# Autodesk Inventor assembly: Second Technological Stage Table Top Assembly
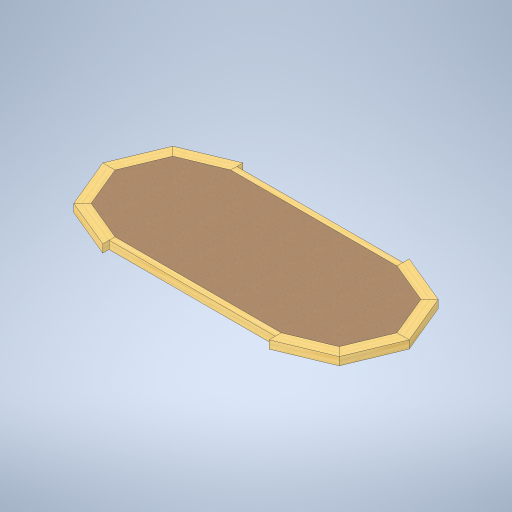
[picture p0: Inventor's stored thumbnail of the model, 512x512]
Saved by Autodesk Inventor 2024 (Build 280153000, 153)
## iProperties
Created: 2020-04-16
Part Number: Second Technological Stage Table Top Assembly
Document SubType Name: Assembly
Designer: SauliusD
Author: SauliusD
## Documents named in this file (4)
- C:\W4INV 2024 Design\PROJECTS\Samples\Composite Material Table\2 Technological Stage Table\Second Technological Stage Table Top Assembly.iam
- C:\W4INV 2024 Design\PROJECTS\Samples\Composite Material Table\2 Technological Stage Table\Round Frame.ipt
- C:\W4INV 2024 Design\PROJECTS\Samples\Composite Material Table\2 Technological Stage Table\Side Insert.ipt
- C:\W4INV 2024 Design\PROJECTS\Samples\Composite Material Table\1 Technolgical stage\First Technolgical stage Table Top Glued Assembly.ipt
## Components (11 placed, 3 different names)
1. Round Frame:1 — Mate:1, Mate:2
2. Side Insert:1
3. First Technolgical stage Table Top Glued Assembly:1 — Flush:1, Flush:2, Flush:3
4. Side Insert:2
5. Round Frame:2
6. Round Frame:3
7. Round Frame:4
8. Round Frame:5 — Mate:1, Mate:2
9. Round Frame:6
10. Round Frame:7
11. Round Frame:8
## Relationships (5: Flush 3, Mate 2)
- Flush:1: First Technolgical stage Table Top Glued Assembly:1
- Flush:2: First Technolgical stage Table Top Glued Assembly:1
- Flush:3: First Technolgical stage Table Top Glued Assembly:1
- Mate:1: Round Frame:1 ↔ Round Frame:5
- Mate:2: Round Frame:1 ↔ Round Frame:5
